# Autodesk Inventor assembly: Ensamblaje_SISTMECANICO_00
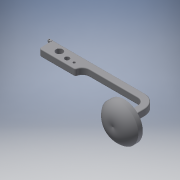
[picture p0: Inventor's stored thumbnail of the model, 180x180]
Saved by Autodesk Inventor 2019.4 (Build 234330000, 330)
## iProperties
Created: 2020-08-24
Part Number: Ensamblaje_SISTMECANICO_00
Document SubType Name: Assembly
Designer: crist
Author: crist
## Documents named in this file (4)
- C:\Users\crist\Desktop\Ensamblaje_SISTMECANICO_00.iam
- C:\Users\crist\Desktop\BALSA_UNDIMOTRIZ\ENSAMBLE_BALSA_UNDIMOTRIZ.iam
- C:\Users\crist\Desktop\BRAZO_UNDIMOTRIZ\EnsamblajE_BRAZO_Y_SUJECIONES.iam
- C:\Users\crist\Desktop\pasador_undimotriz.ipt
## Components (3 placed, 3 different names)
1. ENSAMBLE_BALSA_UNDIMOTRIZ:1 [sub-assembly] — Rígido:1
2. EnsamblajE_BRAZO_Y_SUJECIONES:1 [sub-assembly] — Rígido:1, Rígido:2
3. pasador_undimotriz:1 — Rígido:2
## Relationships (2: WeldJoint 2)
- Rígido:1 [WeldJoint]: ENSAMBLE_BALSA_UNDIMOTRIZ:1 ↔ EnsamblajE_BRAZO_Y_SUJECIONES:1
- Rígido:2 [WeldJoint]: EnsamblajE_BRAZO_Y_SUJECIONES:1 ↔ pasador_undimotriz:1
